# Autodesk Inventor assembly: 001ASM_Base_along
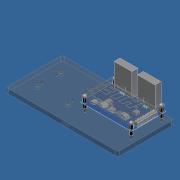
[picture p0: Inventor's stored thumbnail of the model, 180x180]
Saved by Autodesk Inventor 2011 SP1 (Build 150282100, 282)
## iProperties
Created: 2011-09-08
Part Number: 001ASM_Base_along
Document SubType Name: Assembly
Designer: wespep
Author: wespep
## Documents named in this file (6)
- C:\Users\wespep\Documents\RELab\Habtic Paddle\CAD\001ASM_Base_queer.iam
- C:\Users\wespep\Documents\RELab\Habtic Paddle\CAD\Distance_Pin.ipt
- C:\Users\wespep\Documents\RELab\Habtic Paddle\CAD\Platine_Cover.ipt
- C:\Users\wespep\Documents\RELab\Habtic Paddle\CAD\Paddle_Base_queer.ipt
- C:\Users\wespep\Documents\RELab\Habtic Paddle\CAD\MotorAmp\000MotorAmp.iam
- C:\Users\wespep\Documents\Inventor\Content Center Files\R2011\de-DE\ISO 7380\ISO 7380 - M3 x 6.ipt
## Components (15 placed, 5 different names)
1. Paddle_Base_queer:1 — Einfügen:21, Einfügen:22
2. 000MotorAmp:1 [sub-assembly] — Einfügen:5, Einfügen:6, Einfügen:7, Einfügen:8, Einfügen:9, Einfügen:10, Einfügen:19, Einfügen:20
3. Distance_Pin:4 — Einfügen:8, Einfügen:11
4. Platine_Cover:1 — Einfügen:11, Einfügen:12, Einfügen:13, Einfügen:16, Einfügen:17, Einfügen:18
5. Distance_Pin:1 — Einfügen:19
6. Distance_Pin:5 — Einfügen:7
7. Distance_Pin:6 — Einfügen:6
8. Distance_Pin:7 — Einfügen:5, Einfügen:12
9. Distance_Pin:8 — Einfügen:20
10. Distance_Pin:9 — Einfügen:10, Einfügen:22
11. Distance_Pin:10 — Einfügen:9, Einfügen:21
12. ISO 7380 M3 x 6:1 — Einfügen:13
13. ISO 7380 M3 x 6:4 — Einfügen:16
14. ISO 7380 M3 x 6:5 — Einfügen:17
15. ISO 7380 M3 x 6:6 — Einfügen:18
## Relationships (16: Insert 16)
- Einfügen:5 [Insert]: 000MotorAmp:1 ↔ Distance_Pin:7
- Einfügen:6 [Insert]: 000MotorAmp:1 ↔ Distance_Pin:6
- Einfügen:7 [Insert]: 000MotorAmp:1 ↔ Distance_Pin:5
- Einfügen:8 [Insert]: 000MotorAmp:1 ↔ Distance_Pin:4
- Einfügen:9 [Insert]: 000MotorAmp:1 ↔ Distance_Pin:10
- Einfügen:10 [Insert]: 000MotorAmp:1 ↔ Distance_Pin:9
- Einfügen:11 [Insert]: Distance_Pin:4 ↔ Platine_Cover:1
- Einfügen:12 [Insert]: Platine_Cover:1 ↔ Distance_Pin:7
- Einfügen:19 [Insert]: 000MotorAmp:1 ↔ Distance_Pin:1
- Einfügen:20 [Insert]: 000MotorAmp:1 ↔ Distance_Pin:8
- Einfügen:21 [Insert]: Paddle_Base_queer:1 ↔ Distance_Pin:10
- Einfügen:22 [Insert]: Paddle_Base_queer:1 ↔ Distance_Pin:9
- Einfügen:13 [Insert]: Platine_Cover:1 ↔ ISO 7380 M3 x 6:1
- Einfügen:16 [Insert]: Platine_Cover:1 ↔ ISO 7380 M3 x 6:4
- Einfügen:17 [Insert]: Platine_Cover:1 ↔ ISO 7380 M3 x 6:5
- Einfügen:18 [Insert]: Platine_Cover:1 ↔ ISO 7380 M3 x 6:6
